# Autodesk Inventor assembly: Slide_2
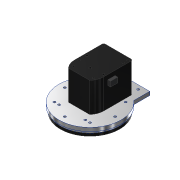
[picture p0: Inventor's stored thumbnail of the model, 180x180]
Saved by Autodesk Inventor 2019 (Build 230136000, 136)
## iProperties
Created: 2018-08-09
Part Number: Slide_2
Document SubType Name: Assembly
Designer: Owner
Mass: 245.828 g
Surface Area: 1925.36 cm^2
Volume: 170.885 cm^3
Density: 1.43855 g/cm^3
Author: Owner
## Documents named in this file (10)
- C:\Users\長谷川翔一\Desktop\キャチロボ2019\ARM2\ARM2\Slide_2_ver2.iam
- C:\Users\長谷川翔一\Desktop\キャチロボ2019\ARM2\ARM2\KRS-4034HV.ipt
- C:\Users\長谷川翔一\Desktop\キャチロボ2019\ARM2\ARM2\ローハイトサーボホーン 2500.ipt
- C:\Users\長谷川翔一\Desktop\キャチロボ2019\ARM2\ARM2\先端モータマウントC.ipt
- C:\Users\長谷川翔一\Desktop\キャチロボ2019\ARM2\ARM2\軸受けワッシャC_ダブルスラスト用(t2_ジュラコン).ipt
- C:\Users\長谷川翔一\Desktop\キャチロボ2019\ARM2\ARM2\出力部品A_ダブルスラスト用(t2_アルミ).ipt
- C:\Users\長谷川翔一\Desktop\キャチロボ2019\ARM2\ARM2\軸受けワッシャA_ダブルスラスト用(t2_ジュラコン).ipt
- C:\Users\長谷川翔一\Desktop\キャチロボ2019\ARM2\ARM2\軸受け用ワッシャD_ダブルスラスト用(t3_ジュラコン).ipt
- C:\Users\長谷川翔一\Desktop\キャチロボ2019\ARM2\ARM2\出力部品B_ダブルスラスト用(t2_アルミ).ipt
- C:\Users\長谷川翔一\Desktop\キャチロボ2019\ARM2\ARM2\軸受けワッシャB_ダブルスラスト用(厚さ2mm_ポケットあり_ジュラコン).ipt
## Components (9 placed, 9 different names)
1. KRS-4034HV:1 — メイト:13, メイト:14, 挿入:11, 挿入:12, 挿入:15, 挿入:16, メイト:17, メイト:26
2. ローハイトサーボホーン 2500:1 — メイト:13, メイト:14, 挿入:21, 挿入:22
3. 先端モータマウントC:1 — 挿入:11, 挿入:12, 挿入:15, 挿入:16, メイト:16, メイト:24, メイト:29
4. 軸受けワッシャC_ダブルスラスト用(t2_ジュラコン):1 — メイト:16, メイト:17
5. 出力部品A_ダブルスラスト用(t2_アルミ):1 — メイト:26, 挿入:17, 挿入:18, 挿入:19, 挿入:20, 挿入:21, 挿入:22
6. 軸受けワッシャA_ダブルスラスト用(t2_ジュラコン):1 — メイト:22, フラッシュ:5, メイト:24, メイト:27, 挿入:23, 挿入:24, 挿入:25
7. 軸受け用ワッシャD_ダブルスラスト用(t3_ジュラコン):1 — メイト:22, フラッシュ:5
8. 出力部品B_ダブルスラスト用(t2_アルミ):1 — 挿入:17, 挿入:18, 挿入:19, 挿入:20, メイト:28
9. 軸受けワッシャB_ダブルスラスト用(厚さ2mm_ポケットあり_ジュラコン):1 — メイト:27, 挿入:23, 挿入:24, 挿入:25, メイト:28, メイト:29
## Relationships (24: Insert 13, Mate 10, Flush 1)
- メイト:13 [Mate]: KRS-4034HV:1 ↔ ローハイトサーボホーン 2500:1
- メイト:14 [Mate]: KRS-4034HV:1 ↔ ローハイトサーボホーン 2500:1
- 挿入:11 [Insert]: KRS-4034HV:1 ↔ 先端モータマウントC:1
- 挿入:12 [Insert]: KRS-4034HV:1 ↔ 先端モータマウントC:1
- 挿入:15 [Insert]: KRS-4034HV:1 ↔ 先端モータマウントC:1
- 挿入:16 [Insert]: KRS-4034HV:1 ↔ 先端モータマウントC:1
- メイト:16 [Mate]: 先端モータマウントC:1 ↔ 軸受けワッシャC_ダブルスラスト用(t2_ジュラコン):1
- メイト:17 [Mate]: KRS-4034HV:1 ↔ 軸受けワッシャC_ダブルスラスト用(t2_ジュラコン):1
- メイト:22 [Mate]: 軸受けワッシャA_ダブルスラスト用(t2_ジュラコン):1 ↔ 軸受け用ワッシャD_ダブルスラスト用(t3_ジュラコン):1
- フラッシュ:5 [Flush]: 軸受けワッシャA_ダブルスラスト用(t2_ジュラコン):1 ↔ 軸受け用ワッシャD_ダブルスラスト用(t3_ジュラコン):1
- メイト:24 [Mate]: 先端モータマウントC:1 ↔ 軸受けワッシャA_ダブルスラスト用(t2_ジュラコン):1
- メイト:26 [Mate]: KRS-4034HV:1 ↔ 出力部品A_ダブルスラスト用(t2_アルミ):1
- メイト:27 [Mate]: 軸受けワッシャA_ダブルスラスト用(t2_ジュラコン):1 ↔ 軸受けワッシャB_ダブルスラスト用(厚さ2mm_ポケットあり_ジュラコン):1
- 挿入:17 [Insert]: 出力部品A_ダブルスラスト用(t2_アルミ):1 ↔ 出力部品B_ダブルスラスト用(t2_アルミ):1
- 挿入:18 [Insert]: 出力部品A_ダブルスラスト用(t2_アルミ):1 ↔ 出力部品B_ダブルスラスト用(t2_アルミ):1
- 挿入:19 [Insert]: 出力部品A_ダブルスラスト用(t2_アルミ):1 ↔ 出力部品B_ダブルスラスト用(t2_アルミ):1
- 挿入:20 [Insert]: 出力部品A_ダブルスラスト用(t2_アルミ):1 ↔ 出力部品B_ダブルスラスト用(t2_アルミ):1
- 挿入:21 [Insert]: ローハイトサーボホーン 2500:1 ↔ 出力部品A_ダブルスラスト用(t2_アルミ):1
- 挿入:22 [Insert]: ローハイトサーボホーン 2500:1 ↔ 出力部品A_ダブルスラスト用(t2_アルミ):1
- 挿入:23 [Insert]: 軸受けワッシャA_ダブルスラスト用(t2_ジュラコン):1 ↔ 軸受けワッシャB_ダブルスラスト用(厚さ2mm_ポケットあり_ジュラコン):1
- 挿入:24 [Insert]: 軸受けワッシャA_ダブルスラスト用(t2_ジュラコン):1 ↔ 軸受けワッシャB_ダブルスラスト用(厚さ2mm_ポケットあり_ジュラコン):1
- 挿入:25 [Insert]: 軸受けワッシャA_ダブルスラスト用(t2_ジュラコン):1 ↔ 軸受けワッシャB_ダブルスラスト用(厚さ2mm_ポケットあり_ジュラコン):1
- メイト:28 [Mate]: 出力部品B_ダブルスラスト用(t2_アルミ):1 ↔ 軸受けワッシャB_ダブルスラスト用(厚さ2mm_ポケットあり_ジュラコン):1
- メイト:29 [Mate]: 先端モータマウントC:1 ↔ 軸受けワッシャB_ダブルスラスト用(厚さ2mm_ポケットあり_ジュラコン):1
